# Autodesk Inventor assembly: UpperArm
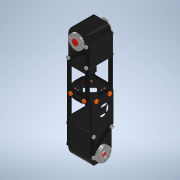
[picture p0: Inventor's stored thumbnail of the model, 180x180]
Saved by Autodesk Inventor 2020 (Build 240168000, 168)
## iProperties
Created: 2021-09-11
Part Number: UpperArm
Document SubType Name: Assembly
Designer: Masato
Mass: 132.402 g
Surface Area: 432.665 cm^2
Volume: 110.152 cm^3
Density: 1.20199 g/cm^3
Author: Masato
## Documents named in this file (9)
- C:\Users\MasatoKubotera\Documents\Inventor\SUSTAINA-OP\UpperBody\Arm\UpperArm.iam
- C:\Users\MasatoKubotera\Documents\Inventor\SUSTAINA-OP\UpperBody\Arm\UpperArm_side_frame.ipt
- C:\Users\MasatoKubotera\Documents\Inventor\SUSTAINA-OP\UpperBody\Arm\UpperArm_diagonal.ipt
- C:\Users\MasatoKubotera\Documents\Inventor\SUSTAINA-OP\ReadyMade\Screw\M2_6-15.ipt
- C:\Users\MasatoKubotera\Documents\Inventor\SUSTAINA-OP\ReadyMade\Screw\M2_6-20.ipt
- C:\Users\MasatoKubotera\Documents\Inventor\SUSTAINA-OP\ReadyMade\Screw\M3-6.ipt
- C:\Users\MasatoKubotera\Documents\Inventor\SUSTAINA-OP\ReadyMade\InsertNut\IRU-304S.ipt
- C:\Users\MasatoKubotera\Documents\Inventor\SUSTAINA-OP\ReadyMade\KONDO\B3M-SC-1040-A_with_ClampHorn_AND_FreeHorn.iam
- C:\Users\MasatoKubotera\Documents\Inventor\SUSTAINA-OP\UpperBody\Arm\UpperArm_side_frame_cloth.ipt
## Components (36 placed, 8 different names)
1. UpperArm_diagonal:1 — 挿入:1, 挿入:2, 挿入:3, 挿入:4, 挿入:5, 挿入:6, 挿入:7, 挿入:8, メイト:3, フラッシュ:1, フラッシュ:2, 挿入:64, 挿入:65, 挿入:66, 挿入:67, 挿入:68, 挿入:69, 挿入:70, 挿入:71
2. UpperArm_side_frame:1 — 挿入:1, 挿入:2, 挿入:32, 挿入:33, 挿入:34, 挿入:74, 挿入:75, 挿入:80, 挿入:84, 挿入:85
3. UpperArm_side_frame:2 — 挿入:3, 挿入:4, 挿入:11, 挿入:12, 挿入:38, 挿入:39, 挿入:40, 挿入:81, 挿入:82, 挿入:83
4. UpperArm_side_frame:3 — 挿入:8, 挿入:7, 挿入:14, 挿入:13, 挿入:35, 挿入:36, 挿入:37, 挿入:77, 挿入:78, 挿入:79
5. UpperArm_side_frame:4 — 挿入:6, 挿入:5, 挿入:15, 挿入:16, 挿入:29, 挿入:30, 挿入:31, 挿入:72, 挿入:73, 挿入:76
6. B3M-SC-1040-A_with_ClampHorn_AND_FreeHorn:1 [sub-assembly] — 挿入:72, 挿入:73, 挿入:76, 挿入:77, 挿入:78, 挿入:79
7. B3M-SC-1040-A_with_ClampHorn_AND_FreeHorn:2 [sub-assembly] — 挿入:74, 挿入:75, 挿入:80, 挿入:81, 挿入:82, 挿入:83
8. UpperArm_side_frame_cloth:1 — 挿入:84, 挿入:85, 挿入:86, 挿入:87
9. M2_6-20:6 — 挿入:40
10. M2_6-20:5 — 挿入:38
11. M2_6-20:4 — 挿入:39
12. M2_6-20:3 — 挿入:37
13. M2_6-20:2 — 挿入:36
14. M2_6-20:1 — 挿入:35
15. M2_6-15:6 — 挿入:34
16. M2_6-15:5 — 挿入:33
17. M2_6-15:4 — 挿入:32
18. M2_6-15:3 — 挿入:31
19. M2_6-15:2 — 挿入:30
20. M2_6-15:1 — 挿入:29
21. M3-6:8 — 挿入:16
22. M3-6:7 — 挿入:15
23. M3-6:6 — 挿入:14
24. M3-6:5 — 挿入:13
25. M3-6:4 — 挿入:12
26. M3-6:3 — 挿入:11
27. M3-6:2 — 挿入:87
28. M3-6:1 — 挿入:86
29. IRU-304S:8 — 挿入:71
30. IRU-304S:7 — 挿入:70
31. IRU-304S:6 — 挿入:69
32. IRU-304S:5 — 挿入:68
33. IRU-304S:4 — 挿入:67
34. IRU-304S:3 — 挿入:66
35. IRU-304S:2 — 挿入:65
36. IRU-304S:1 — 挿入:64
## Relationships (53: Insert 50, Flush 2, Mate 1)
- 挿入:1 [Insert]: UpperArm_diagonal:1 ↔ UpperArm_side_frame:1
- 挿入:2 [Insert]: UpperArm_diagonal:1 ↔ UpperArm_side_frame:1
- 挿入:3 [Insert]: UpperArm_diagonal:1 ↔ UpperArm_side_frame:2
- 挿入:4 [Insert]: UpperArm_diagonal:1 ↔ UpperArm_side_frame:2
- 挿入:5 [Insert]: UpperArm_diagonal:1 ↔ UpperArm_side_frame:4
- 挿入:6 [Insert]: UpperArm_diagonal:1 ↔ UpperArm_side_frame:4
- 挿入:7 [Insert]: UpperArm_diagonal:1 ↔ UpperArm_side_frame:3
- 挿入:8 [Insert]: UpperArm_diagonal:1 ↔ UpperArm_side_frame:3
- 挿入:11 [Insert]: UpperArm_side_frame:2 ↔ M3-6:3
- 挿入:12 [Insert]: UpperArm_side_frame:2 ↔ M3-6:4
- 挿入:13 [Insert]: UpperArm_side_frame:3 ↔ M3-6:5
- 挿入:14 [Insert]: UpperArm_side_frame:3 ↔ M3-6:6
- 挿入:15 [Insert]: UpperArm_side_frame:4 ↔ M3-6:7
- 挿入:16 [Insert]: UpperArm_side_frame:4 ↔ M3-6:8
- 挿入:29 [Insert]: UpperArm_side_frame:4 ↔ M2_6-15:1
- 挿入:30 [Insert]: UpperArm_side_frame:4 ↔ M2_6-15:2
- 挿入:31 [Insert]: UpperArm_side_frame:4 ↔ M2_6-15:3
- 挿入:32 [Insert]: UpperArm_side_frame:1 ↔ M2_6-15:4
- 挿入:33 [Insert]: UpperArm_side_frame:1 ↔ M2_6-15:5
- 挿入:35 [Insert]: UpperArm_side_frame:3 ↔ M2_6-20:1
- 挿入:34 [Insert]: UpperArm_side_frame:1 ↔ M2_6-15:6
- 挿入:36 [Insert]: UpperArm_side_frame:3 ↔ M2_6-20:2
- 挿入:37 [Insert]: UpperArm_side_frame:3 ↔ M2_6-20:3
- 挿入:38 [Insert]: UpperArm_side_frame:2 ↔ M2_6-20:5
- 挿入:39 [Insert]: UpperArm_side_frame:2 ↔ M2_6-20:4
- 挿入:40 [Insert]: UpperArm_side_frame:2 ↔ M2_6-20:6
- メイト:3 [Mate]: UpperArm_diagonal:1
- フラッシュ:1 [Flush]: UpperArm_diagonal:1
- フラッシュ:2 [Flush]: UpperArm_diagonal:1
- 挿入:64 [Insert]: UpperArm_diagonal:1 ↔ IRU-304S:1
- 挿入:65 [Insert]: UpperArm_diagonal:1 ↔ IRU-304S:2
- 挿入:66 [Insert]: UpperArm_diagonal:1 ↔ IRU-304S:3
- 挿入:67 [Insert]: UpperArm_diagonal:1 ↔ IRU-304S:4
- 挿入:68 [Insert]: UpperArm_diagonal:1 ↔ IRU-304S:5
- 挿入:69 [Insert]: UpperArm_diagonal:1 ↔ IRU-304S:6
- 挿入:70 [Insert]: UpperArm_diagonal:1 ↔ IRU-304S:7
- 挿入:71 [Insert]: UpperArm_diagonal:1 ↔ IRU-304S:8
- 挿入:72 [Insert]: UpperArm_side_frame:4 ↔ B3M-SC-1040-A_with_ClampHorn_AND_FreeHorn:1
- 挿入:73 [Insert]: UpperArm_side_frame:4 ↔ B3M-SC-1040-A_with_ClampHorn_AND_FreeHorn:1
- 挿入:74 [Insert]: UpperArm_side_frame:1 ↔ B3M-SC-1040-A_with_ClampHorn_AND_FreeHorn:2
- 挿入:75 [Insert]: UpperArm_side_frame:1 ↔ B3M-SC-1040-A_with_ClampHorn_AND_FreeHorn:2
- 挿入:76 [Insert]: UpperArm_side_frame:4 ↔ B3M-SC-1040-A_with_ClampHorn_AND_FreeHorn:1
- 挿入:77 [Insert]: UpperArm_side_frame:3 ↔ B3M-SC-1040-A_with_ClampHorn_AND_FreeHorn:1
- 挿入:78 [Insert]: UpperArm_side_frame:3 ↔ B3M-SC-1040-A_with_ClampHorn_AND_FreeHorn:1
- 挿入:79 [Insert]: UpperArm_side_frame:3 ↔ B3M-SC-1040-A_with_ClampHorn_AND_FreeHorn:1
- 挿入:80 [Insert]: UpperArm_side_frame:1 ↔ B3M-SC-1040-A_with_ClampHorn_AND_FreeHorn:2
- 挿入:81 [Insert]: UpperArm_side_frame:2 ↔ B3M-SC-1040-A_with_ClampHorn_AND_FreeHorn:2
- 挿入:82 [Insert]: UpperArm_side_frame:2 ↔ B3M-SC-1040-A_with_ClampHorn_AND_FreeHorn:2
- 挿入:83 [Insert]: UpperArm_side_frame:2 ↔ B3M-SC-1040-A_with_ClampHorn_AND_FreeHorn:2
- 挿入:84 [Insert]: UpperArm_side_frame:1 ↔ UpperArm_side_frame_cloth:1
- 挿入:85 [Insert]: UpperArm_side_frame:1 ↔ UpperArm_side_frame_cloth:1
- 挿入:86 [Insert]: UpperArm_side_frame_cloth:1 ↔ M3-6:1
- 挿入:87 [Insert]: UpperArm_side_frame_cloth:1 ↔ M3-6:2
